# Autodesk Inventor assembly: ASY-PRS-DRS 940
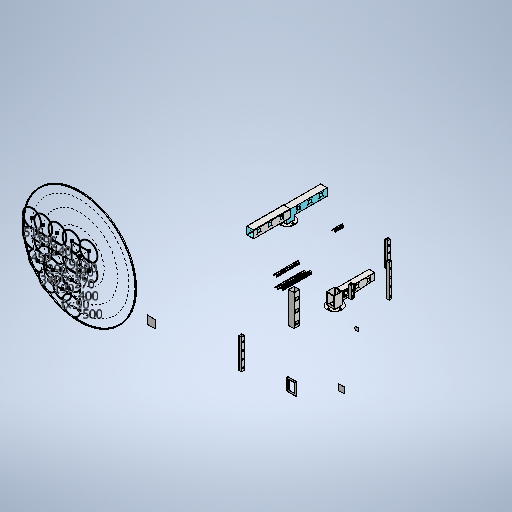
[picture p0: Inventor's stored thumbnail of the model, 512x512]
Saved by Autodesk Inventor 2026.2 (Build 302298010, 298A)
## iProperties
Created: 2026-05-12
Part Number: ASY-PRS-DRS 940
Document SubType Name: Assembly
Designer: admin
Author: admin
## Documents named in this file (25)
- C:\Users\admin\Documents\Inventor\PRS-Purovsk\DRS 940\ASY-PRS-DRS 940.iam
- C:\Users\admin\Documents\Inventor\PRS-Purovsk\PRS-1425 FDS Way FLANGE.ipt
- C:\Users\admin\Documents\Inventor\PRS-Purovsk\ANP 1401 DSB DIMentions.ipt
- C:\Users\admin\Documents\Inventor\PRS-Purovsk\PRS-512 roof 2.ipt
- C:\Users\admin\Documents\Inventor\PRS-Purovsk\PRS-513 roof 3.ipt
- C:\Users\admin\Documents\Inventor\PRS-Purovsk\PRS-513 roof 4.ipt
- C:\Users\admin\Documents\Inventor\PRS-Purovsk\PRS-514 roof 4.ipt
- C:\Users\admin\Documents\Inventor\PRS-Purovsk\PRS-1661 (fds) main way tube.ipt
- C:\Users\admin\Documents\Inventor\PRS-Purovsk\PRS-1662 FDS 1000 way tube 4.ipt
- C:\Users\admin\Documents\Inventor\PRS-Purovsk\PRS-1651 FDS MAIN  FLANGE.ipt
- C:\Users\admin\Documents\Inventor\PRS-Purovsk\PRS-1652 FDS Central tube wall.ipt
- C:\Users\admin\Documents\Inventor\PRS-Purovsk\PRS-1661 FDS 1000 way tube 1.ipt
- C:\Users\admin\Documents\Inventor\PRS-Purovsk\PRS-1662 FDS 1000 way tube 2.ipt
- C:\Users\admin\Documents\Inventor\PRS-Purovsk\PRS-1663 FDS 1200 way tube 3.ipt
- C:\Users\admin\Documents\Inventor\PRS-Purovsk\PRS-1665 FDS 1000 CUP 1.ipt
- C:\Users\admin\Documents\Inventor\PRS-Purovsk\PRS-1666 FDS 1000 CUP 1.ipt
- C:\Users\admin\Documents\Inventor\PRS-Purovsk\PRS-1699 DIM filter-distribution-system 1000.ipt
- C:\Users\admin\Documents\Inventor\PRS-Purovsk\PRS-169859 DIM filter-distribution-system 1000.ipt
- C:\Users\admin\Documents\Inventor\PRS-Purovsk\PRS-1421 FDS Diam way flange 1.ipt
- C:\Users\admin\Documents\Inventor\PRS-Purovsk\PRS-1422 BOTTOM FDS diameter way up.ipt
- C:\Users\admin\Documents\Inventor\PRS-Purovsk\PRS-1423 BOTTOM FDS diameter way down.ipt
- C:\Users\admin\Documents\Inventor\PRS-Purovsk\PRS-1424 FDS diam way cup.ipt
- C:\Users\admin\Documents\Inventor\PRS-Purovsk\PRS-1422 BOTTOM FDS diameter way up_CPY.ipt
- C:\Users\admin\Documents\Inventor\PRS-Purovsk\PRS-1423 BOTTOM FDS diameter way down_CPY.ipt
- C:\Users\admin\Documents\Inventor\PRS-Purovsk\PRS-1651 FDS MAIN  FLANGE_CPY.ipt
## Components (27 placed, 24 different names)
1. PRS-169859 DIM filter-distribution-system 1000:1 — Mate:1, Mate:2, Flush:1
2. PRS-1425 FDS Way FLANGE:1 — Rigid:4
3. ANP 1401 DSB DIMentions:1
4. PRS-512 roof 2:1
5. PRS-513 roof 3:1
6. PRS-513 roof 4:1
7. PRS-514 roof 4:1
8. PRS-1661 (fds) main way tube:1
9. PRS-1662 FDS 1000 way tube 4:1
10. PRS-1651 FDS MAIN  FLANGE:1 — Mate:3
11. PRS-1652 FDS Central tube wall:1 — Rigid:12
12. PRS-1661 FDS 1000 way tube 1:1
13. PRS-1662 FDS 1000 way tube 2:1
14. PRS-1663 FDS 1200 way tube 3:1
15. PRS-1665 FDS 1000 CUP 1:1
16. PRS-1666 FDS 1000 CUP 1:1
17. PRS-1699 DIM filter-distribution-system 1000:1
18. PRS-1421 FDS Diam way flange 1:1
19. PRS-1422 BOTTOM FDS diameter way up:1 — Rigid:13
20. PRS-1423 BOTTOM FDS diameter way down:1 — Rigid:4, Rigid:12, Rigid:13
21. PRS-1424 FDS diam way cup:1
22. PRS-1652 FDS Central tube wall:2 — Mate:3
23. PRS-1422 BOTTOM FDS diameter way up_CPY:1 — Rigid:8
24. PRS-1423 BOTTOM FDS diameter way down_CPY:1 — Rigid:8
25. PRS-1423 BOTTOM FDS diameter way down_CPY:2 — Rigid:9
26. PRS-1422 BOTTOM FDS diameter way up_CPY:2 — Rigid:9
27. PRS-1651 FDS MAIN  FLANGE_CPY:1
## Relationships (9: WeldJoint 5, Mate 3, Flush 1)
- Mate:1: PRS-169859 DIM filter-distribution-system 1000:1
- Mate:2: PRS-169859 DIM filter-distribution-system 1000:1
- Flush:1: PRS-169859 DIM filter-distribution-system 1000:1
- Rigid:4 [WeldJoint]: PRS-1425 FDS Way FLANGE:1 ↔ PRS-1423 BOTTOM FDS diameter way down:1
- Mate:3: PRS-1651 FDS MAIN  FLANGE:1 ↔ PRS-1652 FDS Central tube wall:2
- Rigid:8 [WeldJoint]: PRS-1422 BOTTOM FDS diameter way up_CPY:1 ↔ PRS-1423 BOTTOM FDS diameter way down_CPY:1
- Rigid:9 [WeldJoint]: PRS-1423 BOTTOM FDS diameter way down_CPY:2 ↔ PRS-1422 BOTTOM FDS diameter way up_CPY:2
- Rigid:12 [WeldJoint]: PRS-1652 FDS Central tube wall:1 ↔ PRS-1423 BOTTOM FDS diameter way down:1
- Rigid:13 [WeldJoint]: PRS-1422 BOTTOM FDS diameter way up:1 ↔ PRS-1423 BOTTOM FDS diameter way down:1
